# Autodesk Inventor assembly: EL2-400
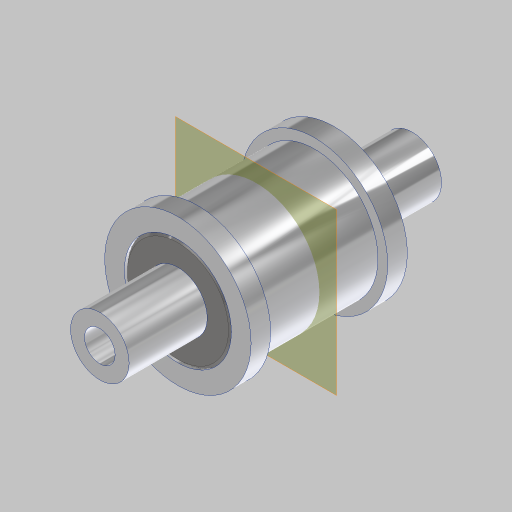
[picture p0: Inventor's stored thumbnail of the model, 512x512]
Saved by Autodesk Inventor 2023.5 (Build 275446000, 446)
## iProperties
Created: 2025-01-11
Part Number: EL2-400
Document SubType Name: Assembly
Designer: mavericks
Author: mavericks
## Documents named in this file (4)
- C:\Users\slick\OneDrive\Desktop\2025-ReefScape---CAD\Elevator\EL2\EL2-400.iam
- C:\Users\slick\OneDrive\Desktop\2025-ReefScape---CAD\Elevator\EL2\EL2-007.ipt
- C:\Users\slick\OneDrive\Desktop\2025-ReefScape---CAD\Elevator\EL2\EL2-008.ipt
- C:\Users\slick\OneDrive\Desktop\2025-ReefScape---CAD\COMMON PARTS\BEARINGS\Ball Bearing 1_4x11_16x5_16 Sealed 1602DC 1602-2RS.ipt
## Components (5 placed, 3 different names)
1. EL2-007:1 — Mate:1, Mate:2, Mate:3, Mate:4, Flush:1, Flush:2, Mate:6
2. EL2-008:1 — Mate:4, Mate:5, Symmetry:1
3. EL2-008:2 — Mate:3, Mate:5, Symmetry:1
4. Ball Bearing 1_4x11_16x5_16 Sealed 1602DC 1602-2RS:1 — Mate:1, Flush:2
5. Ball Bearing 1_4x11_16x5_16 Sealed 1602DC 1602-2RS:2 — Mate:2, Flush:1
## Relationships (9: Mate 6, Flush 2, Symmetry 1)
- Mate:1: EL2-007:1 ↔ Ball Bearing 1_4x11_16x5_16 Sealed 1602DC 1602-2RS:1
- Mate:2: EL2-007:1 ↔ Ball Bearing 1_4x11_16x5_16 Sealed 1602DC 1602-2RS:2
- Mate:3: EL2-007:1 ↔ EL2-008:2
- Mate:4: EL2-007:1 ↔ EL2-008:1
- Flush:1: EL2-007:1 ↔ Ball Bearing 1_4x11_16x5_16 Sealed 1602DC 1602-2RS:2
- Flush:2: EL2-007:1 ↔ Ball Bearing 1_4x11_16x5_16 Sealed 1602DC 1602-2RS:1
- Mate:5: EL2-008:1 ↔ EL2-008:2
- Symmetry:1: EL2-008:1 ↔ EL2-008:2
- Mate:6: EL2-007:1
